# Autodesk Inventor assembly: Case_Pantalla
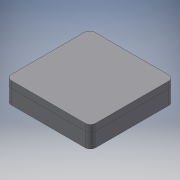
[picture p0: Inventor's stored thumbnail of the model, 180x180]
Saved by Autodesk Inventor 2019 (Build 230136000, 136)
## iProperties
Created: 2018-11-27
Part Number: Case_Pantalla
Document SubType Name: Assembly
Designer: DIEGO 01
Author: DIEGO 01
## Documents named in this file (4)
- C:\Users\CADCAE\Downloads\CAD_thesis\Case_Pantalla.iam
- C:\Users\CADCAE\Downloads\CAD_thesis\Pantalla\Pantalla.ipt
- C:\Users\CADCAE\Downloads\CAD_thesis\Pantalla\case_pantalla_3_inf.ipt
- C:\Users\CADCAE\Downloads\CAD_thesis\Pantalla\case_pantalla_3_sup.ipt
## Components (3 placed, 3 different names)
1. Pantalla:1 — Coincidencia:3, Coincidencia:4, Coincidencia:5
2. case_pantalla_3_inf:1 — Nivelación:1, Nivelación:2, Nivelación:3, Coincidencia:3, Coincidencia:4, Coincidencia:5, Flush:4, Flush:5, Mate:6
3. case_pantalla_3_sup:1 — Flush:4, Flush:5, Mate:6
## Relationships (9: Flush 5, Mate 4)
- Nivelación:1 [Flush]: case_pantalla_3_inf:1
- Nivelación:2 [Flush]: case_pantalla_3_inf:1
- Nivelación:3 [Flush]: case_pantalla_3_inf:1
- Coincidencia:3 [Mate]: Pantalla:1 ↔ case_pantalla_3_inf:1
- Coincidencia:4 [Mate] (0.5 mm): Pantalla:1 ↔ case_pantalla_3_inf:1
- Coincidencia:5 [Mate] (0.5 mm): Pantalla:1 ↔ case_pantalla_3_inf:1
- Flush:4: case_pantalla_3_inf:1 ↔ case_pantalla_3_sup:1
- Flush:5: case_pantalla_3_inf:1 ↔ case_pantalla_3_sup:1
- Mate:6: case_pantalla_3_inf:1 ↔ case_pantalla_3_sup:1
